# Autodesk Inventor assembly: TestAssembly
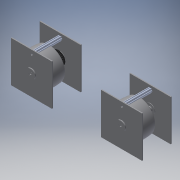
[picture p0: Inventor's stored thumbnail of the model, 180x180]
Saved by Autodesk Inventor 2016 (Build 200138000, 138)
## iProperties
Created: 2017-01-14
Part Number: TestAssembly
Document SubType Name: Assembly
Designer: hamblettk
Author: hamblettk
## Documents named in this file (10)
- F:\FRC\2017\DriveTrainRev2\Individual Parts\TestAssembly.iam
- F:\FRC\2017\DriveTrainRev2\Individual Parts\TestPlate.ipt
- F:\FRC\2017\DriveTrainRev2\Individual Parts\.5Bearing.ipt
- F:\FRC\2017\DriveTrainRev2\Individual Parts\4x2Colson.ipt
- F:\FRC\2017\DriveTrainRev2\Individual Parts\24t9MMPulley6mm.ipt
- F:\FRC\2017\DriveTrainRev2\Individual Parts\24t9MMPulleyExtension.ipt
- F:\FRC\2017\DriveTrainRev2\Individual Parts\3.625Churro.ipt
- F:\FRC\2017\DriveTrainRev2\Individual Parts\3.875Churro.ipt
- F:\FRC\2017\DriveTrainRev2\Individual Parts\.106Spacer.ipt
- F:\FRC\2017\DriveTrainRev2\Individual Parts\.441Spacer.ipt
## Components (21 placed, 9 different names)
1. TestPlate:1 — Mate:1, Mate:2, Flush:1, Mate:18, Flush:3, Flush:4, Mate:23
2. .5Bearing:1 — Mate:1, Mate:2, Mate:6, Mate:20, Flush:2
3. 4x2Colson:1 — Mate:6, Mate:14
4. 24t9MMPulley6mm:1 — Mate:7, Mate:8, Mate:9, Mate:14
5. 24t9MMPulley6mm:2 — Mate:10, Mate:11, Mate:12
6. 24t9MMPulleyExtension:1 — Mate:7, Mate:8, Mate:9, Mate:10, Mate:11, Mate:12
7. TestPlate:2 — Mate:15, Mate:16, Flush:1, Mate:19
8. .5Bearing:2 — Mate:15, Mate:16, Mate:22
9. 3.625Churro:1 — Mate:18, Mate:19
10. 3.875Churro:1 — Mate:20, Flush:2, Mate:21
11. .106Spacer:1 — Mate:21, Mate:22
12. TestPlate:3 — Flush:3, Flush:4, Mate:23, Mate:24, Mate:25, Mate:36
13. .5Bearing:3 — Mate:24, Mate:25, Mate:26, Flush:5, Mate:28
14. 3.875Churro:2 — Mate:26, Flush:5, Mate:27, Mate:32, Mate:37, Mate:39
15. 4x2Colson:2 — Mate:27, Mate:28, Mate:33
16. 24t9MMPulley6mm:3 — Mate:29, Mate:30, Mate:31, Mate:33
17. 24t9MMPulley6mm:4 — Mate:29, Mate:30, Mate:31, Mate:32
18. TestPlate:4 — Mate:34, Mate:35, Mate:38
19. .5Bearing:4 — Mate:34, Mate:35, Mate:37, Mate:40
20. 3.625Churro:2 — Mate:36, Mate:38
21. .441Spacer:1 — Mate:39, Mate:40
## Relationships (40: Mate 35, Flush 5)
- Mate:1: TestPlate:1 ↔ .5Bearing:1
- Mate:2: TestPlate:1 ↔ .5Bearing:1
- Mate:6: .5Bearing:1 ↔ 4x2Colson:1
- Mate:7: 24t9MMPulley6mm:1 ↔ 24t9MMPulleyExtension:1
- Mate:8: 24t9MMPulley6mm:1 ↔ 24t9MMPulleyExtension:1
- Mate:9: 24t9MMPulley6mm:1 ↔ 24t9MMPulleyExtension:1
- Mate:10: 24t9MMPulley6mm:2 ↔ 24t9MMPulleyExtension:1
- Mate:11: 24t9MMPulley6mm:2 ↔ 24t9MMPulleyExtension:1
- Mate:12: 24t9MMPulley6mm:2 ↔ 24t9MMPulleyExtension:1
- Mate:14: 4x2Colson:1 ↔ 24t9MMPulley6mm:1
- Mate:15: TestPlate:2 ↔ .5Bearing:2
- Mate:16: TestPlate:2 ↔ .5Bearing:2
- Flush:1: TestPlate:1 ↔ TestPlate:2
- Mate:18: TestPlate:1 ↔ 3.625Churro:1
- Mate:19: TestPlate:2 ↔ 3.625Churro:1
- Mate:20: .5Bearing:1 ↔ 3.875Churro:1
- Flush:2: .5Bearing:1 ↔ 3.875Churro:1
- Mate:21: 3.875Churro:1 ↔ .106Spacer:1
- Mate:22: .5Bearing:2 ↔ .106Spacer:1
- Flush:3: TestPlate:1 ↔ TestPlate:3
- Flush:4: TestPlate:1 ↔ TestPlate:3
- Mate:23 (152.4 mm): TestPlate:1 ↔ TestPlate:3
- Mate:24: TestPlate:3 ↔ .5Bearing:3
- Mate:25: TestPlate:3 ↔ .5Bearing:3
- Mate:26: .5Bearing:3 ↔ 3.875Churro:2
- Flush:5: .5Bearing:3 ↔ 3.875Churro:2
- Mate:27: 3.875Churro:2 ↔ 4x2Colson:2
- Mate:28: .5Bearing:3 ↔ 4x2Colson:2
- Mate:29: 24t9MMPulley6mm:3 ↔ 24t9MMPulley6mm:4
- Mate:30: 24t9MMPulley6mm:3 ↔ 24t9MMPulley6mm:4
- Mate:31: 24t9MMPulley6mm:3 ↔ 24t9MMPulley6mm:4
- Mate:32: 3.875Churro:2 ↔ 24t9MMPulley6mm:4
- Mate:33: 4x2Colson:2 ↔ 24t9MMPulley6mm:3
- Mate:34: TestPlate:4 ↔ .5Bearing:4
- Mate:35: TestPlate:4 ↔ .5Bearing:4
- Mate:36: TestPlate:3 ↔ 3.625Churro:2
- Mate:37: 3.875Churro:2 ↔ .5Bearing:4
- Mate:38: TestPlate:4 ↔ 3.625Churro:2
- Mate:39: 3.875Churro:2 ↔ .441Spacer:1
- Mate:40: .5Bearing:4 ↔ .441Spacer:1
